# Autodesk Inventor assembly: Rod下
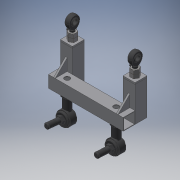
[picture p0: Inventor's stored thumbnail of the model, 180x180]
Saved by Autodesk Inventor 2018 (Build 220112000, 112)
## iProperties
Created: 2017-09-13
Part Number: Rod下
Material: 一般
Document SubType Name: Assembly
Designer: mura5
Author: mura5
## Documents named in this file (8)
- C:\Users\mura5\Documents\RBBR\CAD\サスペンション\上アーム(後).iam
- C:\Users\mura5\Documents\RBBR\CAD\サスペンション\PipeB蓋.ipt
- C:\Users\mura5\Documents\RBBR\CAD\汎用部品\M12_1種ナット.ipt
- C:\Users\mura5\Documents\RBBR\CAD\サスペンション\PipeB(下).ipt
- C:\Users\mura5\Documents\RBBR\CAD\サスペンション\リブ.ipt
- C:\Users\mura5\Documents\RBBR\CAD\サスペンション\アームはり(後).ipt
- C:\Users\mura5\Documents\RBBR\CAD\汎用部品\エルボール14mm\LHSA 14.iam
- C:\Users\mura5\Documents\RBBR\CAD\汎用部品\ピロボール12mm\POS 12.iam
## Components (15 placed, 7 different names)
1. PipeB(下):1 — リジッド:10, フラッシュ:3, メイト:2, フラッシュ:4, メイト:3, メイト:7
2. PipeB蓋:1 — リジッド:2, リジッド:10, リジッド:13
3. M12_1種ナット:1 — リジッド:2, リジッド:3
4. M12_1種ナット:2 — リジッド:3
5. アームはり(後):1 — フラッシュ:1, メイト:1, フラッシュ:3, メイト:2, フラッシュ:4, メイト:3, メイト:4, フラッシュ:5, メイト:6, フラッシュ:6, メイト:8, フラッシュ:7, リジッド:11, リジッド:12
6. PipeB(下):2 — リジッド:9, フラッシュ:1, メイト:1, メイト:4, フラッシュ:5, メイト:5
7. PipeB蓋:2 — リジッド:7, リジッド:9, リジッド:14
8. M12_1種ナット:3 — リジッド:7, リジッド:8
9. M12_1種ナット:4 — リジッド:8
10. リブ:1 — メイト:5, メイト:6, フラッシュ:6
11. リブ:2 — メイト:7, メイト:8, フラッシュ:7
12. LHSA 14:1 [sub-assembly] — リジッド:12
13. LHSA 14:2 [sub-assembly] — リジッド:11
14. POS 12:1 [sub-assembly] — リジッド:13
15. POS 12:2 [sub-assembly] — リジッド:14
## Relationships (24: WeldJoint 10, Mate 8, Flush 6)
- リジッド:2 [WeldJoint]: PipeB蓋:1 ↔ M12_1種ナット:1
- リジッド:3 [WeldJoint]: M12_1種ナット:1 ↔ M12_1種ナット:2
- リジッド:7 [WeldJoint]: PipeB蓋:2 ↔ M12_1種ナット:3
- リジッド:8 [WeldJoint]: M12_1種ナット:3 ↔ M12_1種ナット:4
- リジッド:9 [WeldJoint]: PipeB(下):2 ↔ PipeB蓋:2
- リジッド:10 [WeldJoint]: PipeB(下):1 ↔ PipeB蓋:1
- フラッシュ:1 [Flush]: アームはり(後):1 ↔ PipeB(下):2
- メイト:1 [Mate]: アームはり(後):1 ↔ PipeB(下):2
- フラッシュ:3 [Flush]: PipeB(下):1 ↔ アームはり(後):1
- メイト:2 [Mate]: PipeB(下):1 ↔ アームはり(後):1
- フラッシュ:4 [Flush]: PipeB(下):1 ↔ アームはり(後):1
- メイト:3 [Mate]: PipeB(下):1 ↔ アームはり(後):1
- メイト:4 [Mate]: アームはり(後):1 ↔ PipeB(下):2
- フラッシュ:5 [Flush]: アームはり(後):1 ↔ PipeB(下):2
- メイト:5 [Mate]: PipeB(下):2 ↔ リブ:1
- メイト:6 [Mate]: アームはり(後):1 ↔ リブ:1
- フラッシュ:6 [Flush] (13.75 mm): アームはり(後):1 ↔ リブ:1
- メイト:7 [Mate]: PipeB(下):1 ↔ リブ:2
- メイト:8 [Mate]: アームはり(後):1 ↔ リブ:2
- フラッシュ:7 [Flush] (13.75 mm): アームはり(後):1 ↔ リブ:2
- リジッド:11 [WeldJoint]: アームはり(後):1 ↔ LHSA 14:2
- リジッド:12 [WeldJoint]: アームはり(後):1 ↔ LHSA 14:1
- リジッド:13 [WeldJoint] (10 mm): PipeB蓋:1 ↔ POS 12:1
- リジッド:14 [WeldJoint] (10 mm): PipeB蓋:2 ↔ POS 12:2
